# Autodesk Inventor assembly: KBHandle
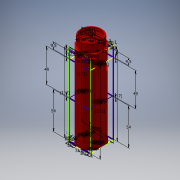
[picture p0: Inventor's stored thumbnail of the model, 180x180]
Saved by Autodesk Inventor 2016 (Build 200138000, 138)
## iProperties
Created: 2014-08-19
Part Number: KBHandle
Document SubType Name: Assembly
Designer: jkao
Author: jkao
## Documents named in this file (4)
- C:\Dropbox\projects\inventor\KBHandle\KBHandle.iam
- C:\Dropbox\projects\inventor\KBHandle\DiffuserCoupler.ipt
- C:\Dropbox\projects\inventor\KBHandle\Handle-Bottom.ipt
- C:\Dropbox\projects\inventor\KBHandle\Handle-Top.ipt
## Components (3 placed, 3 different names)
1. DiffuserCoupler:1 — Flush:2, Flush:3
2. Handle-Bottom:1 — Flush:1, Flush:2
3. Handle-Top:1 — Flush:1, Flush:3
## Relationships (3: Flush 3)
- Flush:1: Handle-Bottom:1 ↔ Handle-Top:1
- Flush:2: DiffuserCoupler:1 ↔ Handle-Bottom:1
- Flush:3: DiffuserCoupler:1 ↔ Handle-Top:1
